# Autodesk Inventor assembly: Full overlay hinge for glass door T7
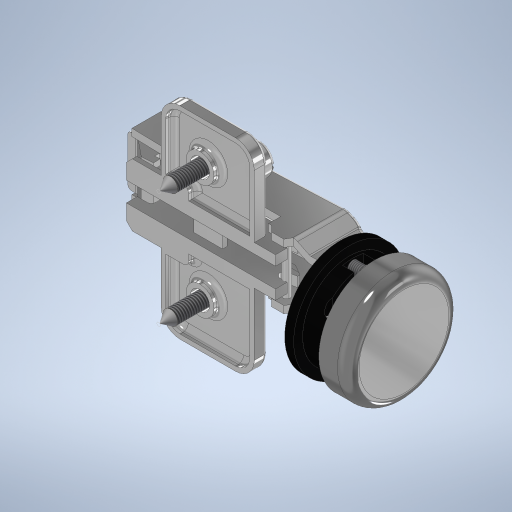
[picture p0: Inventor's stored thumbnail of the model, 512x512]
Saved by Autodesk Inventor 2024 (Build 280153000, 153)
## iProperties
Created: 2014-01-02
Part Number: Full overlay hinge for glass door T7
Document SubType Name: Assembly
Designer: G. Kazokaitis
Author: G. Kazokaitis
## Documents named in this file (8)
- C:\W4INV 2024 Design\_LIBRARY\Hinges\HINGE FOR GLASS PANELS\Full overlay hinge for glass door T7.iam
- C:\W4INV 2024 Design\LIBRARY\Hinges\Parts\Hinge for glass panels\Full overlay hinge case.ipt
- C:\W4INV 2024 Design\LIBRARY\Hinges\Parts\Hinge for glass panels\D26 Linkage.ipt
- C:\W4INV 2024 Design\LIBRARY\Hinges\Parts\Hinge for glass panels\D26 Linkages.ipt
- C:\W4INV 2015 Design\LIBRARY\Hinges\Parts\Hinge for glass panels\Case.ipt
- C:\W4INV 2024 Design\LIBRARY\Hinges\Parts\Hinge for glass panels\Mounting plate.ipt
- C:\W4INV 2024 Design\LIBRARY\Hinges\HINGE FOR GLASS PANELS.iam
- C:\W4INV 2024 Design\_LIBRARY\Hinges\Parts\Hinge for glass panels\Case\Cup glass T7.ipt
## Components (5 placed, 5 different names)
1. Mounting plate:1 — Mate:1, Mate:2, Mate:3, Mate:4, Flush:1, Mate:5
2. Full overlay hinge case:1 — Mate:4, Flush:1, Mate:5, Mate:6, Mate:7, Mate:8, Mate:9, Full overlay opening angle
3. D26 Linkage:1 — Mate:6, Mate:7, Mate:26, Mate:28
4. D26 Linkages:1 — Mate:8, Mate:9, Mate:27
5. Cup glass T7:1 — Mate:26, Mate:27, Mate:28, Full overlay opening angle
## Relationships (14: Mate 12, Flush 1, Angle 1)
- Mate:1: Mounting plate:1
- Mate:2: Mounting plate:1
- Mate:3: Mounting plate:1
- Mate:4 (2.7 mm): Mounting plate:1 ↔ Full overlay hinge case:1
- Flush:1: Mounting plate:1 ↔ Full overlay hinge case:1
- Mate:5 (5.47 mm): Mounting plate:1 ↔ Full overlay hinge case:1
- Mate:6: Full overlay hinge case:1 ↔ D26 Linkage:1
- Mate:7: Full overlay hinge case:1 ↔ D26 Linkage:1
- Mate:8: Full overlay hinge case:1 ↔ D26 Linkages:1
- Mate:9 (1.3 mm): Full overlay hinge case:1 ↔ D26 Linkages:1
- Mate:26: D26 Linkage:1 ↔ Cup glass T7:1
- Mate:27: D26 Linkages:1 ↔ Cup glass T7:1
- Mate:28 (0.35 mm): D26 Linkage:1 ↔ Cup glass T7:1
- Full overlay opening angle [Angle] (90 deg): Full overlay hinge case:1 ↔ Cup glass T7:1
## Named parameters: Edge_distance = 37 mm
